# Autodesk Inventor assembly: Extruder Assembly
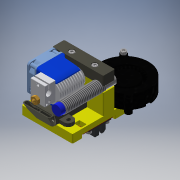
[picture p0: Inventor's stored thumbnail of the model, 180x180]
Saved by Autodesk Inventor 2016 (Build 200138000, 138)
## iProperties
Created: 2017-03-19
Part Number: Extruder Assembly
Document SubType Name: Assembly
Designer: Scott
Author: Scott
## Documents named in this file (11)
- E:\Scott Projects\3D Printing\CoreXY\Extruder Assembly.iam
- E:\Scott Projects\3D Printing\CoreXY\Extruder Mount.ipt
- E:\Scott Projects\3D Printing\CoreXY\Workspaces\Workspace\E3D V6 Hotend.iam
- E:\Scott Projects\3D Printing\CoreXY\Radial-Cooling-Fan-5015-DC12V.iam
- E:\Scott Projects\3D Printing\CoreXY\Duct v5.ipt
- E:\Scott Projects\3D Printing\CoreXY\Endstop_Opto_TCST2103.iam
- E:\Scott Projects\3D Printing\CoreXY\LJ12A3-4-Z Sensor.ipt
- C:\Users\Scott\Documents\Inventor\Content Center Files\R2016\en-US\AS 1420\AS 1420 - 1973 - M3 x 8.ipt
- E:\Scott Projects\3D Printing\CoreXY\Retainer.ipt
- C:\Users\Scott\Documents\Inventor\Content Center Files\R2016\en-US\AS 1420\AS 1420 - 1973 - M3 x 14.ipt
- C:\Users\Scott\Documents\Inventor\Content Center Files\R2016\en-US\AS 1420\AS 1420 - 1973 - M3 x 20.ipt
## Components (15 placed, 10 different names)
1. Extruder Mount:1 — Mate:1, Mate:3, Mate:4, Mate:6, Mate:8, Mate:9, Mate:10, Mate:11, Mate:12, Mate:13, Mate:14, Mate:15, Flush:4, Flush:5, Mate:16, Mate:17, Insert:9, Angle:1
2. Radial-Cooling-Fan-5015-DC12V:1 [sub-assembly] — Mate:1, Mate:16, Insert:8
3. Duct v5:1 — Mate:3, Mate:4
4. Endstop_Opto_TCST2103:1 [sub-assembly] — Mate:6, Mate:10, Mate:11, Insert:2, Insert:3
5. LJ12A3-4-Z Sensor:1 — Mate:8, Mate:9
6. Endstop_Opto_TCST2103:2 [sub-assembly] — Mate:12, Mate:13, Mate:14, Insert:4, Insert:5
7. AS 1420 - Metric M3 x 8:1 — Insert:3
8. AS 1420 - Metric M3 x 8:2 — Insert:2
9. AS 1420 - Metric M3 x 8:3 — Insert:4
10. AS 1420 - Metric M3 x 8:4 — Insert:5
11. Retainer:1 — Mate:15, Flush:4, Flush:5, Insert:6, Insert:7
12. AS 1420 - Metric M3 x 14:1 — Insert:6
13. AS 1420 - Metric M3 x 14:2 — Insert:7
14. AS 1420 - Metric M3 x 20:1 — Insert:8
15. E3D V6 Hotend:1 [sub-assembly] — Mate:17, Insert:9, Angle:1
## Relationships (25: Mate 14, Insert 8, Flush 2, Angle 1)
- Mate:1: Extruder Mount:1 ↔ Radial-Cooling-Fan-5015-DC12V:1
- Mate:3: Extruder Mount:1 ↔ Duct v5:1
- Mate:4: Extruder Mount:1 ↔ Duct v5:1
- Mate:6: Extruder Mount:1 ↔ Endstop_Opto_TCST2103:1
- Mate:8 (-3 mm): Extruder Mount:1 ↔ LJ12A3-4-Z Sensor:1
- Mate:9 (-6 mm): Extruder Mount:1 ↔ LJ12A3-4-Z Sensor:1
- Mate:10: Extruder Mount:1 ↔ Endstop_Opto_TCST2103:1
- Mate:11: Extruder Mount:1 ↔ Endstop_Opto_TCST2103:1
- Mate:12: Extruder Mount:1 ↔ Endstop_Opto_TCST2103:2
- Mate:13: Extruder Mount:1 ↔ Endstop_Opto_TCST2103:2
- Mate:14: Extruder Mount:1 ↔ Endstop_Opto_TCST2103:2
- Insert:2: Endstop_Opto_TCST2103:1 ↔ AS 1420 - Metric M3 x 8:2
- Insert:3: Endstop_Opto_TCST2103:1 ↔ AS 1420 - Metric M3 x 8:1
- Insert:4: Endstop_Opto_TCST2103:2 ↔ AS 1420 - Metric M3 x 8:3
- Insert:5: Endstop_Opto_TCST2103:2 ↔ AS 1420 - Metric M3 x 8:4
- Mate:15: Extruder Mount:1 ↔ Retainer:1
- Flush:4: Extruder Mount:1 ↔ Retainer:1
- Flush:5: Extruder Mount:1 ↔ Retainer:1
- Mate:16: Extruder Mount:1 ↔ Radial-Cooling-Fan-5015-DC12V:1
- Insert:6: Retainer:1 ↔ AS 1420 - Metric M3 x 14:1
- Insert:7: Retainer:1 ↔ AS 1420 - Metric M3 x 14:2
- Insert:8: Radial-Cooling-Fan-5015-DC12V:1 ↔ AS 1420 - Metric M3 x 20:1
- Mate:17: Extruder Mount:1 ↔ E3D V6 Hotend:1
- Insert:9 (0.25 mm): Extruder Mount:1 ↔ E3D V6 Hotend:1
- Angle:1 (0 deg): Extruder Mount:1 ↔ E3D V6 Hotend:1
